# Autodesk Inventor assembly: Manipulator
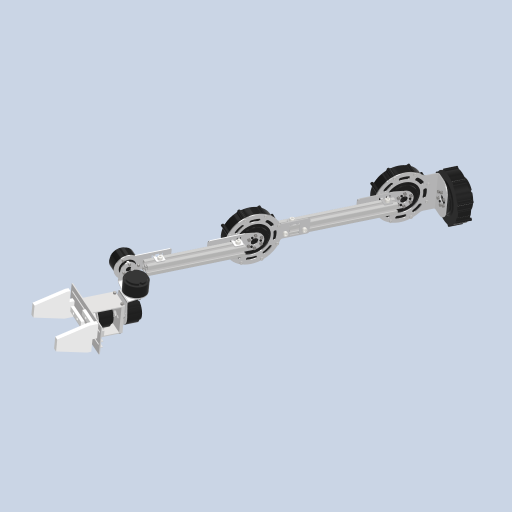
[picture p0: Inventor's stored thumbnail of the model, 512x512]
Saved by Autodesk Inventor 2023 (Build 270158000, 158)
## iProperties
Created: 2024-11-08
Part Number: Manipulator
Document SubType Name: Assembly
Designer: kiyo
Mass: 1528.92 g
Surface Area: 2699.84 cm^2
Volume: 487.593 cm^3
Density: 3.13566 g/cm^3
Author: kiyo
## Documents named in this file (21)
- D:\GitHub\inventor\syu-si\OfficeRobot\Manipulator\Manipulator.iam
- D:\GitHub\inventor\syu-si\OfficeRobot\ReadyMade\Steadywin\GIM8108-8.iam
- D:\GitHub\inventor\syu-si\OfficeRobot\Manipulator\elbow-pitch-bracket.ipt
- D:\GitHub\inventor\syu-si\OfficeRobot\ReadyMade\Screw\M3_6mm.ipt
- D:\GitHub\inventor\syu-si\OfficeRobot\ReadyMade\Steadywin\GIM3505-8_with-driver.ipt
- D:\GitHub\inventor\syu-si\OfficeRobot\Manipulator\wrist_roll_plate.ipt
- D:\GitHub\inventor\syu-si\OfficeRobot\Manipulator\wrist-pitch-plate.ipt
- D:\GitHub\inventor\syu-si\OfficeRobot\ReadyMade\Screw\M2-5_6mm.ipt
- D:\GitHub\inventor\syu-si\OfficeRobot\ReadyMade\Screw\CBSH3-8.ipt
- D:\GitHub\inventor\syu-si\OfficeRobot\ReadyMade\Screw\FWSJJ-D5-V2_6-T4_5.ipt
- D:\GitHub\inventor\syu-si\OfficeRobot\ReadyMade\Screw\M2-5_10mm.ipt
- D:\GitHub\inventor\syu-si\OfficeRobot\ReadyMade\Screw\HNTU5-5.ipt
- D:\GitHub\inventor\syu-si\OfficeRobot\Manipulator\pitch_plate_20mm.ipt
- D:\GitHub\inventor\syu-si\OfficeRobot\Manipulator\sholder_roll_bracket.ipt
- D:\GitHub\inventor\syu-si\OfficeRobot\ReadyMade\Screw\SCB5-22.ipt
- D:\GitHub\inventor\syu-si\OfficeRobot\ReadyMade\Screw\SCB5-8.ipt
- D:\GitHub\inventor\syu-si\OfficeRobot\Manipulator\Hand_tyokudou.iam
- D:\GitHub\inventor\syu-si\OfficeRobot\Manipulator\wrist-yaw-plate.ipt
- D:\GitHub\inventor\syu-si\OfficeRobot\ReadyMade\Aluminum-frame\NFS5-2020-200-AV15-BV180.ipt
- D:\GitHub\inventor\syu-si\OfficeRobot\ReadyMade\Aluminum-frame\NFS5-2020-170-AV15-BV145.ipt
- D:\GitHub\inventor\syu-si\OfficeRobot\table_kan.ipt
## Components (99 placed, 20 different names)
1. sholder_roll_bracket:1 — 挿入:350, 挿入:361, 挿入:362, 挿入:363, 挿入:364, 挿入:365, 挿入:366, 挿入:414, フラッシュ:5, 挿入:492, 挿入:493
2. wrist-yaw-plate:1 — 挿入:456, 挿入:457, 挿入:458, 挿入:485
3. wrist_roll_plate:2 — 挿入:402, 挿入:403, 挿入:404, 挿入:405, 挿入:406, 挿入:407, 挿入:485, 挿入:486
4. Hand_tyokudou:1 [sub-assembly] — 挿入:487, 挿入:488, 挿入:489, 挿入:490, 角度:59, 角度:60, フラッシュ:3, メイト:98, フラッシュ:4
5. pitch_plate_20mm:1 — 挿入:465, 正接:44, メイト:62, 角度:74, 角度:75, 正接:45, メイト:65, メイト:79, 正接:53, 挿入:479, 挿入:480, 挿入:481, 挿入:482, 挿入:483, 挿入:484, 正接:66, 角度:87
6. HNTU5-5:30 — 角度:75
7. SCB5-8:15 — 正接:45, メイト:65
8. elbow-pitch-bracket:1 — 挿入:467, 挿入:468, メイト:81, 正接:55, メイト:85, 正接:57, メイト:87, 正接:58
9. pitch_plate_20mm:2 — 挿入:469, メイト:89, 正接:59, 正接:60, 角度:80, 角度:82, 角度:83, 正接:64, メイト:95, 正接:67
10. wrist-pitch-plate:1 — メイト:70, メイト:71, メイト:72, 正接:46, 正接:47, 正接:48, 正接:49, 角度:76, 角度:77, 角度:78, 正接:50, 正接:51, 挿入:470, 挿入:471, 挿入:494, 挿入:495, 挿入:496
11. NFS5-2020-200-AV15-BV180:1
12. HNTU5-5:31
13. SCB5-22:9 — メイト:79, 正接:53
14. HNTU5-5:32
15. SCB5-22:10 — メイト:81, 正接:55
16. HNTU5-5:33
17. SCB5-8:16 — メイト:85, 正接:57
18. HNTU5-5:34
19. SCB5-8:17 — メイト:87, 正接:58
20. HNTU5-5:35 — 角度:80
21. SCB5-22:11 — メイト:89, 正接:59, 正接:60
22. NFS5-2020-170-AV15-BV145:1 — 角度:86, メイト:99, メイト:100
23. HNTU5-5:36 — 角度:83
24. SCB5-8:18 — 正接:64, メイト:95
25. table_kan:1 — フラッシュ:5
26. HNTU5-5:37 — 角度:86, メイト:99, メイト:100
27. SCB5-8:19 — 正接:67
28. M2-5_6mm:16 — 挿入:494
29. M2-5_6mm:17 — 挿入:496
30. M2-5_6mm:18 — 挿入:495
31. M3_6mm:1 — 挿入:337
32. M3_6mm:2 — 挿入:336
33. M3_6mm:3 — 挿入:334
34. M3_6mm:4 — 挿入:338
35. M3_6mm:5 — 挿入:339
36. M3_6mm:6 — 挿入:335
37. M3_6mm:7 — 挿入:481
38. M3_6mm:8 — 挿入:482
39. M3_6mm:9 — 挿入:484
40. M3_6mm:10 — 挿入:483
41. M3_6mm:11 — 挿入:480
42. M3_6mm:12 — 挿入:479
43. M3_6mm:13 — 挿入:361
44. M3_6mm:14 — 挿入:363
45. M3_6mm:15 — 挿入:362
46. M3_6mm:16 — 挿入:364
47. M3_6mm:17 — 挿入:365
48. M3_6mm:18 — 挿入:366
49. CBSH3-8:1 — 挿入:307
50. CBSH3-8:2 — 挿入:308
51. CBSH3-8:3 — 挿入:302, 挿入:492
52. CBSH3-8:4 — 挿入:304
53. CBSH3-8:5 — 挿入:309
54. CBSH3-8:6 — 挿入:303
55. CBSH3-8:7 — 挿入:305
56. CBSH3-8:8 — 挿入:306
57. CBSH3-8:9 — 挿入:332
58. CBSH3-8:10 — 挿入:327, 挿入:468
59. CBSH3-8:11 — 挿入:330
60. CBSH3-8:12 — 挿入:328
61. CBSH3-8:13 — 挿入:329
62. CBSH3-8:14 — 挿入:331
63. CBSH3-8:15 — 挿入:326
64. CBSH3-8:16 — 挿入:333
65. M2-5_6mm:13
66. M2-5_6mm:14
67. M2-5_6mm:15
68. M2-5_10mm:7 — 挿入:402
69. M2-5_10mm:8 — 挿入:403
70. M2-5_10mm:9 — 挿入:404
71. M2-5_10mm:10 — 挿入:430
72. M2-5_10mm:11
73. M2-5_10mm:12
74. M2-5_10mm:13 — 挿入:453, 挿入:456
75. M2-5_10mm:15 — 挿入:454, 挿入:457
76. M2-5_10mm:14 — 挿入:455, 挿入:458
77. FWSJJ-D5-V2_6-T4_5:16 — 挿入:454
78. FWSJJ-D5-V2_6-T4_5:17 — 挿入:453
79. FWSJJ-D5-V2_6-T4_5:18 — 挿入:455
80. FWSJJ-D5-V2_6-T4_5:10 — 挿入:407
81. FWSJJ-D5-V2_6-T4_5:11 — 挿入:405
82. FWSJJ-D5-V2_6-T4_5:12 — 挿入:406
83. FWSJJ-D5-V2_6-T4_5:13 — 挿入:430, 挿入:487
84. FWSJJ-D5-V2_6-T4_5:14 — 挿入:489
85. FWSJJ-D5-V2_6-T4_5:15 — 挿入:488
86. HNTU5-5:22 — 挿入:412, 角度:76
87. SCB5-8:8 — 挿入:412, メイト:72, 正接:49, 正接:50
88. HNTU5-5:23 — 挿入:411, 角度:77
89. SCB5-8:9 — 挿入:411, メイト:71, 正接:48, 正接:51
90. SCB5-22:8 — 挿入:375, メイト:70, 正接:46, 正接:47
91. SCB5-8:7 — 正接:44, メイト:62
92. HNTU5-5:14 — 挿入:375, 角度:78
93. HNTU5-5:21 — 角度:74
94. GIM8108-8:1 [sub-assembly] — 挿入:350, 肩ピッチとの角度関係, 環境固定, 環境固定2
95. GIM8108-8:2 [sub-assembly] — 挿入:302, 挿入:303, 挿入:304, 挿入:305, 挿入:306, 挿入:307, 挿入:308, 挿入:309, 挿入:414, 肩ピッチとの角度関係, 挿入:465, 挿入:493, 角度:87
96. GIM8108-8:3 [sub-assembly] — 挿入:326, 挿入:327, 挿入:328, 挿入:329, 挿入:330, 挿入:331, 挿入:332, 挿入:333, 挿入:334, 挿入:335, 挿入:336, 挿入:337, 挿入:338, 挿入:339, 挿入:467, 挿入:469, 角度:82
97. GIM3505-8_with-driver:9 — 挿入:470, 挿入:471, 挿入:486
98. GIM3505-8_with-driver:8
99. GIM3505-8_with-driver:10 — 挿入:490
## Relationships (156: Insert 87, Mate 29, Tangent 21, Angle 16, Flush 3)
- 挿入:302 [Insert] (2 mm): CBSH3-8:3 ↔ GIM8108-8:2
- 挿入:303 [Insert] (2 mm): CBSH3-8:6 ↔ GIM8108-8:2
- 挿入:304 [Insert] (2 mm): CBSH3-8:4 ↔ GIM8108-8:2
- 挿入:305 [Insert] (2 mm): CBSH3-8:7 ↔ GIM8108-8:2
- 挿入:306 [Insert] (2 mm): CBSH3-8:8 ↔ GIM8108-8:2
- 挿入:307 [Insert] (2 mm): CBSH3-8:1 ↔ GIM8108-8:2
- 挿入:308 [Insert] (2 mm): CBSH3-8:2 ↔ GIM8108-8:2
- 挿入:309 [Insert] (2 mm): CBSH3-8:5 ↔ GIM8108-8:2
- 挿入:326 [Insert] (2 mm): CBSH3-8:15 ↔ GIM8108-8:3
- 挿入:327 [Insert] (2 mm): CBSH3-8:10 ↔ GIM8108-8:3
- 挿入:328 [Insert] (2 mm): CBSH3-8:12 ↔ GIM8108-8:3
- 挿入:329 [Insert] (2 mm): CBSH3-8:13 ↔ GIM8108-8:3
- 挿入:330 [Insert] (2 mm): CBSH3-8:11 ↔ GIM8108-8:3
- 挿入:331 [Insert] (2 mm): CBSH3-8:14 ↔ GIM8108-8:3
- 挿入:332 [Insert] (2 mm): CBSH3-8:9 ↔ GIM8108-8:3
- 挿入:333 [Insert] (2 mm): CBSH3-8:16 ↔ GIM8108-8:3
- 挿入:334 [Insert] (2 mm): M3_6mm:3 ↔ GIM8108-8:3
- 挿入:335 [Insert] (2 mm): M3_6mm:6 ↔ GIM8108-8:3
- 挿入:336 [Insert] (2 mm): M3_6mm:2 ↔ GIM8108-8:3
- 挿入:337 [Insert] (2 mm): M3_6mm:1 ↔ GIM8108-8:3
- 挿入:338 [Insert] (2 mm): M3_6mm:4 ↔ GIM8108-8:3
- 挿入:339 [Insert] (2 mm): M3_6mm:5 ↔ GIM8108-8:3
- 挿入:350 [Insert]: sholder_roll_bracket:1 ↔ GIM8108-8:1
- 挿入:361 [Insert]: sholder_roll_bracket:1 ↔ M3_6mm:13
- 挿入:362 [Insert]: sholder_roll_bracket:1 ↔ M3_6mm:15
- 挿入:363 [Insert]: sholder_roll_bracket:1 ↔ M3_6mm:14
- 挿入:364 [Insert]: sholder_roll_bracket:1 ↔ M3_6mm:16
- 挿入:365 [Insert]: sholder_roll_bracket:1 ↔ M3_6mm:17
- 挿入:366 [Insert]: sholder_roll_bracket:1 ↔ M3_6mm:18
- 挿入:375 [Insert] (-1.2 mm): SCB5-22:8 ↔ HNTU5-5:14
- [Insert] (3.2 mm): SCB5-8:7 ↔ HNTU5-5:21
- [Insert]: wrist_roll_plate:2 ↔ M2-5_6mm:13
- [Insert]: wrist_roll_plate:2 ↔ M2-5_6mm:14
- [Insert]: wrist_roll_plate:2 ↔ M2-5_6mm:15
- [Insert]: wrist_roll_plate:2 ↔ GIM3505-8_with-driver:8
- [Insert]: wrist_roll_plate:2 ↔ GIM3505-8_with-driver:8
- 挿入:402 [Insert]: wrist_roll_plate:2 ↔ M2-5_10mm:7
- 挿入:403 [Insert]: wrist_roll_plate:2 ↔ M2-5_10mm:8
- 挿入:404 [Insert]: wrist_roll_plate:2 ↔ M2-5_10mm:9
- 挿入:405 [Insert]: wrist_roll_plate:2 ↔ FWSJJ-D5-V2_6-T4_5:11
- 挿入:406 [Insert]: wrist_roll_plate:2 ↔ FWSJJ-D5-V2_6-T4_5:12
- 挿入:407 [Insert]: wrist_roll_plate:2 ↔ FWSJJ-D5-V2_6-T4_5:10
- 挿入:411 [Insert] (3.2 mm): HNTU5-5:23 ↔ SCB5-8:9
- 挿入:412 [Insert] (3.2 mm): HNTU5-5:22 ↔ SCB5-8:8
- 挿入:414 [Insert]: sholder_roll_bracket:1 ↔ GIM8108-8:2
- 挿入:430 [Insert] (2 mm): M2-5_10mm:10 ↔ FWSJJ-D5-V2_6-T4_5:13
- [Insert] (2 mm): M2-5_10mm:11 ↔ FWSJJ-D5-V2_6-T4_5:14
- [Insert] (2 mm): M2-5_10mm:12 ↔ FWSJJ-D5-V2_6-T4_5:15
- 挿入:453 [Insert] (2 mm): M2-5_10mm:13 ↔ FWSJJ-D5-V2_6-T4_5:17
- 挿入:454 [Insert] (2 mm): M2-5_10mm:15 ↔ FWSJJ-D5-V2_6-T4_5:16
- 挿入:455 [Insert] (2 mm): M2-5_10mm:14 ↔ FWSJJ-D5-V2_6-T4_5:18
- 挿入:456 [Insert]: wrist-yaw-plate:1 ↔ M2-5_10mm:13
- 挿入:457 [Insert]: wrist-yaw-plate:1 ↔ M2-5_10mm:15
- 挿入:458 [Insert]: wrist-yaw-plate:1 ↔ M2-5_10mm:14
- [Insert]: wrist-yaw-plate:1 ↔ GIM3505-8_with-driver:10
- [Insert]: wrist-yaw-plate:1 ↔ GIM3505-8_with-driver:10
- 肩ピッチとの角度関係 [Angle] (0 deg): GIM8108-8:1 ↔ GIM8108-8:2
- 環境固定 [Angle] (-90 deg): GIM8108-8:1
- 挿入:465 [Insert]: pitch_plate_20mm:1 ↔ GIM8108-8:2
- 正接:44 [Tangent] (0.25 mm): pitch_plate_20mm:1 ↔ SCB5-8:7
- メイト:62 [Mate]: pitch_plate_20mm:1 ↔ SCB5-8:7
- 角度:74 [Angle] (0 deg): pitch_plate_20mm:1 ↔ HNTU5-5:21
- [Insert] (3.2 mm): HNTU5-5:30 ↔ SCB5-8:15
- 角度:75 [Angle] (0 deg): pitch_plate_20mm:1 ↔ HNTU5-5:30
- 正接:45 [Tangent] (0.25 mm): pitch_plate_20mm:1 ↔ SCB5-8:15
- メイト:65 [Mate]: pitch_plate_20mm:1 ↔ SCB5-8:15
- 挿入:467 [Insert]: elbow-pitch-bracket:1 ↔ GIM8108-8:3
- 挿入:468 [Insert]: elbow-pitch-bracket:1 ↔ CBSH3-8:10
- 挿入:469 [Insert]: pitch_plate_20mm:2 ↔ GIM8108-8:3
- メイト:70 [Mate]: wrist-pitch-plate:1 ↔ SCB5-22:8
- メイト:71 [Mate]: wrist-pitch-plate:1 ↔ SCB5-8:9
- メイト:72 [Mate]: wrist-pitch-plate:1 ↔ SCB5-8:8
- 正接:46 [Tangent] (0.25 mm): wrist-pitch-plate:1 ↔ SCB5-22:8
- 正接:47 [Tangent] (7.5 mm): wrist-pitch-plate:1 ↔ SCB5-22:8
- 正接:48 [Tangent] (0.25 mm): wrist-pitch-plate:1 ↔ SCB5-8:9
- 正接:49 [Tangent] (0.25 mm): wrist-pitch-plate:1 ↔ SCB5-8:8
- 角度:76 [Angle] (0 deg): wrist-pitch-plate:1 ↔ HNTU5-5:22
- 角度:77 [Angle] (0 deg): wrist-pitch-plate:1 ↔ HNTU5-5:23
- 角度:78 [Angle] (0 deg): wrist-pitch-plate:1 ↔ HNTU5-5:14
- 正接:50 [Tangent] (7.5 mm): wrist-pitch-plate:1 ↔ SCB5-8:8
- 正接:51 [Tangent] (7.5 mm): wrist-pitch-plate:1 ↔ SCB5-8:9
- 挿入:470 [Insert]: wrist-pitch-plate:1 ↔ GIM3505-8_with-driver:9
- 挿入:471 [Insert]: wrist-pitch-plate:1 ↔ GIM3505-8_with-driver:9
- [Mate]: pitch_plate_20mm:1 ↔ NFS5-2020-200-AV15-BV180:1
- [Mate]: pitch_plate_20mm:1 ↔ NFS5-2020-200-AV15-BV180:1
- [Mate] (1 mm): HNTU5-5:30 ↔ NFS5-2020-200-AV15-BV180:1
- [Mate] (1 mm): NFS5-2020-200-AV15-BV180:1 ↔ HNTU5-5:21
- [Insert] (-1.2 mm): HNTU5-5:31 ↔ SCB5-22:9
- メイト:79 [Mate]: pitch_plate_20mm:1 ↔ SCB5-22:9
- 正接:53 [Tangent] (0.25 mm): pitch_plate_20mm:1 ↔ SCB5-22:9
- [Mate] (1 mm): NFS5-2020-200-AV15-BV180:1 ↔ HNTU5-5:31
- [Tangent] (12.5 mm): NFS5-2020-200-AV15-BV180:1 ↔ SCB5-22:9
- [Insert] (-1.2 mm): HNTU5-5:32 ↔ SCB5-22:10
- メイト:81 [Mate]: elbow-pitch-bracket:1 ↔ SCB5-22:10
- 正接:55 [Tangent] (0.25 mm): elbow-pitch-bracket:1 ↔ SCB5-22:10
- [Mate] (1 mm): NFS5-2020-200-AV15-BV180:1 ↔ HNTU5-5:32
- [Mate]: elbow-pitch-bracket:1 ↔ NFS5-2020-200-AV15-BV180:1
- [Mate]: elbow-pitch-bracket:1 ↔ NFS5-2020-200-AV15-BV180:1
- [Tangent] (17.5 mm): NFS5-2020-200-AV15-BV180:1 ↔ SCB5-22:10
- [Insert] (3.2 mm): HNTU5-5:33 ↔ SCB5-8:16
- メイト:85 [Mate]: elbow-pitch-bracket:1 ↔ SCB5-8:16
- [Angle] (0 deg): NFS5-2020-200-AV15-BV180:1 ↔ HNTU5-5:33
- 正接:57 [Tangent] (0.25 mm): elbow-pitch-bracket:1 ↔ SCB5-8:16
- [Mate] (1 mm): NFS5-2020-200-AV15-BV180:1 ↔ HNTU5-5:33
- [Insert] (3.2 mm): HNTU5-5:34 ↔ SCB5-8:17
- メイト:87 [Mate]: elbow-pitch-bracket:1 ↔ SCB5-8:17
- 正接:58 [Tangent] (0.25 mm): elbow-pitch-bracket:1 ↔ SCB5-8:17
- [Mate] (1 mm): NFS5-2020-200-AV15-BV180:1 ↔ HNTU5-5:34
- [Insert] (-1.2 mm): HNTU5-5:35 ↔ SCB5-22:11
- メイト:89 [Mate]: pitch_plate_20mm:2 ↔ SCB5-22:11
- 正接:59 [Tangent] (0.25 mm): pitch_plate_20mm:2 ↔ SCB5-22:11
- 正接:60 [Tangent] (7.5 mm): pitch_plate_20mm:2 ↔ SCB5-22:11
- 角度:80 [Angle] (0 deg): pitch_plate_20mm:2 ↔ HNTU5-5:35
- [Mate]: pitch_plate_20mm:2 ↔ NFS5-2020-170-AV15-BV145:1
- [Mate]: pitch_plate_20mm:2 ↔ NFS5-2020-170-AV15-BV145:1
- [Tangent] (7.5 mm): SCB5-22:11 ↔ NFS5-2020-170-AV15-BV145:1
- [Mate]: wrist-pitch-plate:1 ↔ NFS5-2020-170-AV15-BV145:1
- [Mate]: wrist-pitch-plate:1 ↔ NFS5-2020-170-AV15-BV145:1
- [Tangent] (22.5 mm): NFS5-2020-170-AV15-BV145:1 ↔ SCB5-22:8
- 角度:82 [Angle] (0 deg): pitch_plate_20mm:2 ↔ GIM8108-8:3
- [Insert] (3.2 mm): HNTU5-5:36 ↔ SCB5-8:18
- 角度:83 [Angle] (0 deg): pitch_plate_20mm:2 ↔ HNTU5-5:36
- 正接:64 [Tangent] (0.25 mm): pitch_plate_20mm:2 ↔ SCB5-8:18
- メイト:95 [Mate]: pitch_plate_20mm:2 ↔ SCB5-8:18
- [Mate] (1 mm): NFS5-2020-170-AV15-BV145:1 ↔ HNTU5-5:36
- 挿入:479 [Insert]: pitch_plate_20mm:1 ↔ M3_6mm:12
- 挿入:480 [Insert]: pitch_plate_20mm:1 ↔ M3_6mm:11
- 挿入:481 [Insert]: pitch_plate_20mm:1 ↔ M3_6mm:7
- 挿入:482 [Insert]: pitch_plate_20mm:1 ↔ M3_6mm:8
- 挿入:483 [Insert]: pitch_plate_20mm:1 ↔ M3_6mm:10
- 挿入:484 [Insert]: pitch_plate_20mm:1 ↔ M3_6mm:9
- 挿入:485 [Insert] (4.5 mm): wrist-yaw-plate:1 ↔ wrist_roll_plate:2
- 挿入:486 [Insert] (4.5 mm): wrist_roll_plate:2 ↔ GIM3505-8_with-driver:9
- 挿入:487 [Insert]: Hand_tyokudou:1 ↔ FWSJJ-D5-V2_6-T4_5:13
- 挿入:488 [Insert]: Hand_tyokudou:1 ↔ FWSJJ-D5-V2_6-T4_5:15
- 挿入:489 [Insert]: Hand_tyokudou:1 ↔ FWSJJ-D5-V2_6-T4_5:14
- 挿入:490 [Insert] (4.5 mm): Hand_tyokudou:1 ↔ GIM3505-8_with-driver:10
- 角度:59 [Angle] (0 deg): Hand_tyokudou:1
- 角度:60 [Angle] (0 deg): Hand_tyokudou:1
- フラッシュ:3 [Flush] (250 mm): Hand_tyokudou:1
- メイト:98 [Mate]: Hand_tyokudou:1
- フラッシュ:4 [Flush]: Hand_tyokudou:1
- フラッシュ:5 [Flush]: sholder_roll_bracket:1 ↔ table_kan:1
- 正接:66 [Tangent] (-16.5 mm): pitch_plate_20mm:1
- 環境固定2 [Angle] (0 deg): GIM8108-8:1
- [Insert] (3.2 mm): HNTU5-5:37 ↔ SCB5-8:19
- 角度:86 [Angle] (0 deg): NFS5-2020-170-AV15-BV145:1 ↔ HNTU5-5:37
- メイト:99 [Mate]: NFS5-2020-170-AV15-BV145:1 ↔ HNTU5-5:37
- メイト:100 [Mate] (1 mm): NFS5-2020-170-AV15-BV145:1 ↔ HNTU5-5:37
- 正接:67 [Tangent] (0.25 mm): pitch_plate_20mm:2 ↔ SCB5-8:19
- 挿入:492 [Insert]: sholder_roll_bracket:1 ↔ CBSH3-8:3
- 挿入:493 [Insert]: sholder_roll_bracket:1 ↔ GIM8108-8:2
- 角度:87 [Angle] (0 deg): pitch_plate_20mm:1 ↔ GIM8108-8:2
- 挿入:494 [Insert]: wrist-pitch-plate:1 ↔ M2-5_6mm:16
- 挿入:495 [Insert]: wrist-pitch-plate:1 ↔ M2-5_6mm:18
- 挿入:496 [Insert]: wrist-pitch-plate:1 ↔ M2-5_6mm:17
## Named parameters: d492_d466 = 3.2 mm, d516_d512 = 0 mm, d517_d513 = 0 mm, d519_d268 = 0 mm, d520_d269 = 0 mm, d521_d270 = 0 mm, d583_d581 = 2 mm, d584_d581 = 2 mm, d733_d492_d466 = 3.2 mm, d770_d470 = -1.2 mm, d775_d470 = -1.2 mm, d782_d733_d492_d466 = 3.2 mm, d787_d782_d733_d492_d466 = 3.2 mm, d791_d770_d470 = -1.2 mm, d804_d733_d492_d466 = 3.2 mm, d850_d804_d733_d492_d466 = 3.2 mm
